# Autodesk Inventor assembly: Steering Assembly
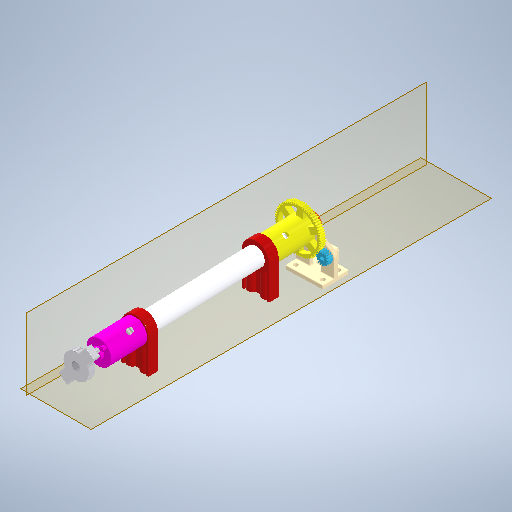
[picture p0: Inventor's stored thumbnail of the model, 512x512]
Saved by Autodesk Inventor 2025.2 (Build 292293000, 293)
## iProperties
Created: 2025-02-05
Part Number: Steering Assembly
Document SubType Name: Assembly
Designer: eason
Author: eason
## Documents named in this file (10)
- C:\Users\eason\Desktop\Code\Unojoy-Simulator-Rig\CAD\Steering\Steering Assembly.iam
- C:\Users\eason\Desktop\Code\Unojoy-Simulator-Rig\CAD\Steering\Steering Back.ipt
- C:\Users\eason\Desktop\Code\Unojoy-Simulator-Rig\CAD\Steering\Steering Front.ipt
- C:\Users\eason\Desktop\Code\Unojoy-Simulator-Rig\CAD\Steering\Steering Gear.ipt
- C:\Users\eason\Desktop\Code\Unojoy-Simulator-Rig\CAD\Steering\Steering Mounting Plate.ipt
- C:\Users\eason\Desktop\Code\Unojoy-Simulator-Rig\CAD\Steering\Steering PVC.ipt
- C:\Users\eason\Desktop\Code\Unojoy-Simulator-Rig\CAD\Steering\Steering Support.ipt
- C:\Users\eason\Desktop\Code\Unojoy-Simulator-Rig\CAD\Steering\Encoder Gear.ipt
- C:\Users\eason\Desktop\Code\Unojoy-Simulator-Rig\CAD\Steering\Steering Gear Plate.ipt
- C:\Users\eason\Desktop\Code\Unojoy-Simulator-Rig\CAD\Steering\Locating Pin.ipt
## Components (11 placed, 9 different names)
1. Steering Back:1 — Cylindrical:3, Mate:5, Angle:1, Mate:12, Insert:5
2. Steering Front:1 — Angle:1, Insert:5
3. Steering Mounting Plate:1 — Mate:8, Insert:2, Insert:3
4. Steering PVC:1 — Cylindrical:3, Mate:5, Cylindrical:6, Cylindrical:7, Insert:1, Mate:13, Cylindrical:8, Cylindrical:9
5. Steering Support:1 — Mate:10, Cylindrical:6, Mate:14
6. Steering Support:2 — Mate:11, Cylindrical:7, Mate:12
7. Spur Gear1:1 — Insert:3
8. Spur Gear2:1 — Insert:1, Mate:13, Mate:14, Insert:2, Insert:4, Mate:15, Mate:16
9. Steering Gear Plate:1 — Insert:4, Mate:15, Mate:16
10. Locating Pin:1 — Cylindrical:9
11. Locating Pin:2 — Cylindrical:8
## Relationships (20: Mate 9, CylindricalJoint 5, Insert 5, Angle 1)
- Cylindrical:3: Steering Back:1 ↔ Steering PVC:1
- Mate:5: Steering Back:1 ↔ Steering PVC:1
- Angle:1 (0 deg): Steering Back:1 ↔ Steering Front:1
- Mate:8: Steering Mounting Plate:1
- Mate:10: Steering Support:1
- Mate:11: Steering Support:2
- Cylindrical:6: Steering PVC:1 ↔ Steering Support:1
- Cylindrical:7: Steering PVC:1 ↔ Steering Support:2
- Mate:12: Steering Back:1 ↔ Steering Support:2
- Insert:1: Steering PVC:1 ↔ Spur Gear2:1
- Mate:13: Steering PVC:1 ↔ Spur Gear2:1
- Mate:14: Steering Support:1 ↔ Spur Gear2:1
- Insert:2: Steering Mounting Plate:1 ↔ Spur Gear2:1
- Insert:3: Steering Mounting Plate:1 ↔ Spur Gear1:1
- Insert:4: Spur Gear2:1 ↔ Steering Gear Plate:1
- Mate:15: Spur Gear2:1 ↔ Steering Gear Plate:1
- Mate:16: Spur Gear2:1 ↔ Steering Gear Plate:1
- Insert:5 (-30 mm): Steering Back:1 ↔ Steering Front:1
- Cylindrical:8: Steering PVC:1 ↔ Locating Pin:2
- Cylindrical:9: Steering PVC:1 ↔ Locating Pin:1
